# Autodesk Inventor assembly: HPTBD5-SEP
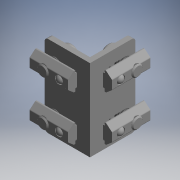
[picture p0: Inventor's stored thumbnail of the model, 180x180]
Saved by Autodesk Inventor 2017.3 (Build 213256000, 256)
## iProperties
Category: PARTsolutions
Company: MISUMI
Part Number: HPTBD5-SEP
Catalog Web Link: www.cadenas.de
Description: HPTBS5, SHPTBS5, HPTBD5, SHPTBD5, HPTBDW5, SHPTBDW5, HPTGS5-Sheet Metal Brackets - For HFS5 Series - Bent Type
Vendor: MISUMI
Document SubType Name: Assembly
Designer: partserver
Manufacturer: MISUMI
Mass: 5.83413 g
Surface Area: 63.0691 cm^2
Volume: 5.83413 cm^3
Density: 1 g/cm^3
Title: HPTBD5-SEP
Author: Cadenas PARTsolutions
Comments: Sheet Metal Brackets - For HFS5 Series - Bent Type
PSOL_IDENT_0: {$CADENAS_DATA\23d-libs\misumi\metric\38_al_extrusions_blackets\5\hptbs5_asmtab.prj},245 {VTYP=3D},{
PSOL_IDENT_1: STYP=ASSTAB},{NB=HPTBD5-SEP},{LINA=HPTBD5-SEP},{NN=HPTBS5, SHPTBS5, HPTBD5, SHPTBD5, HPTBDW5, SHPTBD
PSOL_IDENT_2: W5, HPTGS5},{DATE=08.06.2021 08:25:19},{GEOMDATE=03.04.2020 02:15:02},{VERSION=},{LINEID=270},{WBVAR=
PSOL_IDENT_3: MAT,SHPT,NOH,ALT1},{WBNUMERIC=}  {NB=HPTBD5-SEP},{LINA=HPTBD5-SEP},{KT=5},{PN=HPTBD5-SEP},{TYPE=HPTB
PSOL_IDENT_4: D},{NO=5},{MAT=},{ST=Trivalent Chromate},{SHPT=L},{SHPTALG= 'L', 'L-Shaped Bent','B', 'Both Ends Bem
PSOL_IDENT_5: t' },{NOH=BD},{NOHALG= 'BS','2','BD','4','BDW','8' },{MASS=21},{T=2.3},{ALT1=-SEP},{AB=CBM5-8},{NOB=
PSOL_IDENT_6: 4},{AN=HNTP5-5},{NON=4},{AB1=5-8},{AN1=5-5},{MAT1='', 'Low Carbon Steel', 'S', '304 Stainless Steel'
PSOL_IDENT_7: },{PPATH=hptbs5/hptbs5_asmtpl.prj}
NB: HPTBD5-SEP
NN: HPTBS5, SHPTBS5, HPTBD5, SHPTBD5, HPTBDW5, SHPTBDW5, HPTGS5
NT: Sheet Metal Brackets - For HFS5 Series - Bent Type
NBSYN: $PN.
LINA: HPTBD5-SEP
CATALOG: Misumi
PN: HPTBD5-SEP
NO: 5
MAT: Low Carbon Steel
ST: Trivalent Chromate
SHPT: L-Shaped Bent
NOH: 4
MASS: 21
T: 2.3
ALT1: with SEP (Post-Assembly Fitting Spring Nuts Set of Applicable Bolt and Nut)
AB: CBM5-8
NOB: 4
AN: HNTP5-5
NON: 4
SUPPLIER: MISUMI
ARTICLENO: HPTBD5-SEP
BOMINFO: HPTBD5-SEP
CREATOR: CADENAS GmbH
## Documents named in this file (4)
- e:\temp\worker_2\temp\exporttempdir_3244_92_EUDIF\format_0\HPTBD5-SEP.iam
- e:\temp\worker_2\temp\exporttempdir_3244_92_EUDIF\format_0\HPTBD5-SEP_b_.ipt
- e:\temp\worker_2\temp\exporttempdir_3244_92_EUDIF\format_0\CBM5-8.ipt
- e:\temp\worker_2\temp\exporttempdir_3244_92_EUDIF\format_0\HNTP5-5.ipt
## Components (9 placed, 3 different names)
1. HPTBD5-SEP_b_:1 — to_cbm_1_1_XY@1 <-> bolt_XY@2, to_cbm_1_1_Z@1 <-> bolt_Z@2, to_cbm_1_1_YZ@1 <-> bolt_YZ@2, to_cbm_1_2_XY@1 <-> bolt_XY@3, to_cbm_1_2_Z@1 <-> bolt_Z@3, to_cbm_1_2_YZ@1 <-> bolt_YZ@3, to_cbm_2_1_XY@1 <-> bolt_XY@4, to_cbm_2_1_Z@1 <-> bolt_Z@4, to_cbm_2_1_YZ@1 <-> bolt_YZ@4, to_cbm_2_2_XY@1 <-> bolt_XY@5, to_cbm_2_2_Z@1 <-> bolt_Z@5, to_cbm_2_2_YZ@1 <-> bolt_YZ@5, to_hntp5_1_1_XY@1 <-> to_frames_XY@6, to_hntp5_1_1_Z@1 <-> to_frames_Z@6, to_hntp5_1_1_YZ@1 <-> to_frames_YZ@6, to_hntp5_1_2_XY@1 <-> to_frames_XY@7, to_hntp5_1_2_Z@1 <-> to_frames_Z@7, to_hntp5_1_2_YZ@1 <-> to_frames_YZ@7, to_hntp5_2_1_XY@1 <-> to_frames_XY@8, to_hntp5_2_1_Z@1 <-> to_frames_Z@8, to_hntp5_2_1_YZ@1 <-> to_frames_YZ@8, to_hntp5_2_2_XY@1 <-> to_frames_XY@9, to_hntp5_2_2_Z@1 <-> to_frames_Z@9, to_hntp5_2_2_YZ@1 <-> to_frames_YZ@9
2. CBM5-8:1 — to_cbm_1_1_XY@1 <-> bolt_XY@2, to_cbm_1_1_Z@1 <-> bolt_Z@2, to_cbm_1_1_YZ@1 <-> bolt_YZ@2
3. CBM5-8:2 — to_cbm_1_2_XY@1 <-> bolt_XY@3, to_cbm_1_2_Z@1 <-> bolt_Z@3, to_cbm_1_2_YZ@1 <-> bolt_YZ@3
4. CBM5-8:3 — to_cbm_2_1_XY@1 <-> bolt_XY@4, to_cbm_2_1_Z@1 <-> bolt_Z@4, to_cbm_2_1_YZ@1 <-> bolt_YZ@4
5. CBM5-8:4 — to_cbm_2_2_XY@1 <-> bolt_XY@5, to_cbm_2_2_Z@1 <-> bolt_Z@5, to_cbm_2_2_YZ@1 <-> bolt_YZ@5
6. HNTP5-5:1 — to_hntp5_1_1_XY@1 <-> to_frames_XY@6, to_hntp5_1_1_Z@1 <-> to_frames_Z@6, to_hntp5_1_1_YZ@1 <-> to_frames_YZ@6
7. HNTP5-5:2 — to_hntp5_1_2_XY@1 <-> to_frames_XY@7, to_hntp5_1_2_Z@1 <-> to_frames_Z@7, to_hntp5_1_2_YZ@1 <-> to_frames_YZ@7
8. HNTP5-5:3 — to_hntp5_2_1_XY@1 <-> to_frames_XY@8, to_hntp5_2_1_Z@1 <-> to_frames_Z@8, to_hntp5_2_1_YZ@1 <-> to_frames_YZ@8
9. HNTP5-5:4 — to_hntp5_2_2_XY@1 <-> to_frames_XY@9, to_hntp5_2_2_Z@1 <-> to_frames_Z@9, to_hntp5_2_2_YZ@1 <-> to_frames_YZ@9
## Relationships (24: Mate 16, Angle 8)
- to_cbm_1_1_XY@1 <-> bolt_XY@2 [Mate]: HPTBD5-SEP_b_:1 ↔ CBM5-8:1
- to_cbm_1_1_Z@1 <-> bolt_Z@2 [Mate]: HPTBD5-SEP_b_:1 ↔ CBM5-8:1
- to_cbm_1_1_YZ@1 <-> bolt_YZ@2 [Angle] (0 deg): HPTBD5-SEP_b_:1 ↔ CBM5-8:1
- to_cbm_1_2_XY@1 <-> bolt_XY@3 [Mate]: HPTBD5-SEP_b_:1 ↔ CBM5-8:2
- to_cbm_1_2_Z@1 <-> bolt_Z@3 [Mate]: HPTBD5-SEP_b_:1 ↔ CBM5-8:2
- to_cbm_1_2_YZ@1 <-> bolt_YZ@3 [Angle] (0 deg): HPTBD5-SEP_b_:1 ↔ CBM5-8:2
- to_cbm_2_1_XY@1 <-> bolt_XY@4 [Mate]: HPTBD5-SEP_b_:1 ↔ CBM5-8:3
- to_cbm_2_1_Z@1 <-> bolt_Z@4 [Mate]: HPTBD5-SEP_b_:1 ↔ CBM5-8:3
- to_cbm_2_1_YZ@1 <-> bolt_YZ@4 [Angle] (0 deg): HPTBD5-SEP_b_:1 ↔ CBM5-8:3
- to_cbm_2_2_XY@1 <-> bolt_XY@5 [Mate]: HPTBD5-SEP_b_:1 ↔ CBM5-8:4
- to_cbm_2_2_Z@1 <-> bolt_Z@5 [Mate]: HPTBD5-SEP_b_:1 ↔ CBM5-8:4
- to_cbm_2_2_YZ@1 <-> bolt_YZ@5 [Angle] (0 deg): HPTBD5-SEP_b_:1 ↔ CBM5-8:4
- to_hntp5_1_1_XY@1 <-> to_frames_XY@6 [Mate]: HPTBD5-SEP_b_:1 ↔ HNTP5-5:1
- to_hntp5_1_1_Z@1 <-> to_frames_Z@6 [Mate]: HPTBD5-SEP_b_:1 ↔ HNTP5-5:1
- to_hntp5_1_1_YZ@1 <-> to_frames_YZ@6 [Angle] (0 deg): HPTBD5-SEP_b_:1 ↔ HNTP5-5:1
- to_hntp5_1_2_XY@1 <-> to_frames_XY@7 [Mate]: HPTBD5-SEP_b_:1 ↔ HNTP5-5:2
- to_hntp5_1_2_Z@1 <-> to_frames_Z@7 [Mate]: HPTBD5-SEP_b_:1 ↔ HNTP5-5:2
- to_hntp5_1_2_YZ@1 <-> to_frames_YZ@7 [Angle] (0 deg): HPTBD5-SEP_b_:1 ↔ HNTP5-5:2
- to_hntp5_2_1_XY@1 <-> to_frames_XY@8 [Mate]: HPTBD5-SEP_b_:1 ↔ HNTP5-5:3
- to_hntp5_2_1_Z@1 <-> to_frames_Z@8 [Mate]: HPTBD5-SEP_b_:1 ↔ HNTP5-5:3
- to_hntp5_2_1_YZ@1 <-> to_frames_YZ@8 [Angle] (0 deg): HPTBD5-SEP_b_:1 ↔ HNTP5-5:3
- to_hntp5_2_2_XY@1 <-> to_frames_XY@9 [Mate]: HPTBD5-SEP_b_:1 ↔ HNTP5-5:4
- to_hntp5_2_2_Z@1 <-> to_frames_Z@9 [Mate]: HPTBD5-SEP_b_:1 ↔ HNTP5-5:4
- to_hntp5_2_2_YZ@1 <-> to_frames_YZ@9 [Angle] (0 deg): HPTBD5-SEP_b_:1 ↔ HNTP5-5:4
